# Autodesk Inventor assembly: E3Dv5
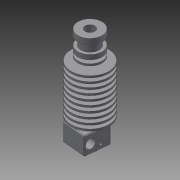
[picture p0: Inventor's stored thumbnail of the model, 180x180]
Saved by Autodesk Inventor 2014 (Build 180170000, 170)
## iProperties
Created: 2014-09-30
Part Number: E3Dv5
Document SubType Name: Assembly
Designer: ThatOtherGuy
Author: ThatOtherGuy
## Documents named in this file (6)
- U:\Hobbies\Inventor\KosselCNC1515\Hotend\E3Dv5.iam
- U:\Hobbies\Inventor\KosselCNC1515\Hotend\E3D_Chamber.ipt
- U:\Hobbies\Inventor\KosselCNC1515\Hotend\E3D_Heat_Break.ipt
- U:\Hobbies\Inventor\KosselCNC1515\Hotend\E3D_Heaterblock.ipt
- U:\Hobbies\Inventor\Content Center Files\R2014\en-US\ANSI B18.3.6M(01)\ANSI B18.3.6M - M3x0.5 x 5(2).ipt
- U:\Hobbies\Inventor\KosselCNC1515\Hotend\E3D_Nozzle.ipt
## Components (5 placed, 5 different names)
1. E3D_Chamber:1 — Insert:1
2. E3D_Heat_Break:1 — Insert:1, Insert:2
3. E3D_Heaterblock:1 — Mate:1, Flush:1, Insert:2, Insert:3
4. Broached Hexagon Socket Set Screw - Flat Point - Metric M3x0.5 x 5:1 — Mate:1, Flush:1
5. E3D_Nozzle:1 — Insert:3
## Relationships (5: Insert 3, Mate 1, Flush 1)
- Insert:1 (-17 mm): E3D_Chamber:1 ↔ E3D_Heat_Break:1
- Mate:1: E3D_Heaterblock:1 ↔ Broached Hexagon Socket Set Screw - Flat Point - Metric M3x0.5 x 5:1
- Flush:1 (-1.5 mm): E3D_Heaterblock:1 ↔ Broached Hexagon Socket Set Screw - Flat Point - Metric M3x0.5 x 5:1
- Insert:2 (-5 mm): E3D_Heat_Break:1 ↔ E3D_Heaterblock:1
- Insert:3 (-7 mm): E3D_Heaterblock:1 ↔ E3D_Nozzle:1
